# Autodesk Inventor assembly: NeckAssembly
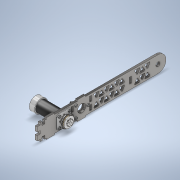
[picture p0: Inventor's stored thumbnail of the model, 180x180]
Saved by Autodesk Inventor 2022 (Build 260153000, 153)
## iProperties
Created: 2021-05-22
Part Number: NeckAssembly
Document SubType Name: Assembly
Designer: M3rob
Mass: 10239.7 g
Surface Area: 3396.39 cm^2
Volume: 1644.12 cm^3
Density: 6.22807 g/cm^3
Author: M3rob
## Documents named in this file (10)
- C:\Users\M3rob\Documents\GrabCAD\FireBird 250 Pound Gaming Machine\Drafts\FrameDrafts\Draft_04\Assemblies\NeckAssembly.iam
- C:\Users\M3rob\Documents\GrabCAD\FireBird 250 Pound Gaming Machine\Drafts\FrameDrafts\Draft_04\Chassis and Mounting\NeckFrame_Draft04.ipt
- C:\Users\M3rob\Documents\GrabCAD\FireBird 250 Pound Gaming Machine\Drafts\FrameDrafts\Draft_04\Chassis and Mounting\MotorMountingPlate_Draft02.ipt
- C:\Users\M3rob\Documents\GrabCAD\FireBird 250 Pound Gaming Machine\Drafts\FrameDrafts\Draft_04\Electronics\MagMotorMockup.ipt
- C:\Users\M3rob\Documents\GrabCAD\FireBird 250 Pound Gaming Machine\Drafts\FrameDrafts\Draft_04\Hardware\92620A656_GeneralChassisScrew.ipt
- C:\Users\M3rob\Documents\GrabCAD\FireBird 250 Pound Gaming Machine\Drafts\FrameDrafts\Draft_04\Hardware\94895A815_GeneralChassisNut.ipt
- C:\Users\M3rob\Documents\GrabCAD\FireBird 250 Pound Gaming Machine\Drafts\FrameDrafts\Draft_04\Hardware\2737T262_JackshaftSprocket_Modified.ipt
- C:\Users\M3rob\Documents\GrabCAD\FireBird 250 Pound Gaming Machine\Drafts\FrameDrafts\Draft_04\Weapon System\6524K421_TorqueLimiter.ipt
- C:\Users\M3rob\Documents\GrabCAD\FireBird 250 Pound Gaming Machine\Drafts\FrameDrafts\Draft_04\Hardware\91253A198_WeaponMotorMountingScrew.ipt
- C:\Users\M3rob\Documents\GrabCAD\FireBird 250 Pound Gaming Machine\Drafts\FrameDrafts\Draft_04\Weapon System\JackShaftRetentionPlate.ipt
## Components (24 placed, 9 different names)
1. NeckFrame_Draft04:1 — Mate:1, Mate:2, Mate:3, Mate:4, Mate:5, Mate:29, Mate:30, Mate:31, Mate:32, Mate:46, Mate:47, Mate:48, Mate:49, Mate:50, Mate:51, Mate:52
2. MotorMountingPlate_Draft02:1 — Mate:1, Mate:2, Mate:3, Mate:4, Mate:5, Mate:6, Mate:7, Mate:8, Mate:17, Mate:18, Mate:19, Mate:20, Mate:21, Mate:22, Mate:23, Mate:24, Mate:36, Mate:37, Mate:38, Mate:39, Flush:1, Flush:2, Flush:3, Flush:4, Mate:42
3. MagMotorMockup:1 — Mate:6, Mate:7, Mate:8, Mate:35
4. 92620A656_GeneralChassisScrew:1 — Mate:20, Mate:22, Mate:27
5. 94895A815_GeneralChassisNut:1 — Mate:28, Mate:29
6. 92620A656_GeneralChassisScrew:2 — Mate:19, Mate:21, Mate:25
7. 94895A815_GeneralChassisNut:2 — Mate:25, Mate:31
8. 92620A656_GeneralChassisScrew:3 — Mate:18, Mate:24, Mate:28
9. 94895A815_GeneralChassisNut:3 — Mate:27, Mate:30
10. 92620A656_GeneralChassisScrew:4 — Mate:17, Mate:23, Mate:26
11. 94895A815_GeneralChassisNut:4 — Mate:26, Mate:32
12. 2737T262_JackshaftSprocket_Modified:1 — Mate:34
13. 6524K421_TorqueLimiter:1 — Mate:34, Mate:35, Mate:42
14. 91253A198_WeaponMotorMountingScrew:1 — Mate:36, Flush:4
15. 91253A198_WeaponMotorMountingScrew:2 — Mate:37, Flush:3
16. 91253A198_WeaponMotorMountingScrew:3 — Mate:39, Flush:2
17. 91253A198_WeaponMotorMountingScrew:4 — Mate:38, Flush:1
18. JackShaftRetentionPlate:1 — Mate:46, Mate:47, Mate:48, Mate:49, Mate:53, Mate:54, Mate:55, Mate:56
19. 94895A815_GeneralChassisNut:5 — Flush:5, Flush:6
20. 92620A656_GeneralChassisScrew:5 — Mate:52, Mate:54
21. 94895A815_GeneralChassisNut:6 — Flush:5, Mate:56
22. 92620A656_GeneralChassisScrew:6 — Mate:51, Mate:55
23. 94895A815_GeneralChassisNut:7 — Flush:6
24. 92620A656_GeneralChassisScrew:7 — Mate:50, Mate:53
## Relationships (52: Mate 46, Flush 6)
- Mate:1: NeckFrame_Draft04:1 ↔ MotorMountingPlate_Draft02:1
- Mate:2: NeckFrame_Draft04:1 ↔ MotorMountingPlate_Draft02:1
- Mate:3: NeckFrame_Draft04:1 ↔ MotorMountingPlate_Draft02:1
- Mate:4: NeckFrame_Draft04:1 ↔ MotorMountingPlate_Draft02:1
- Mate:5: NeckFrame_Draft04:1 ↔ MotorMountingPlate_Draft02:1
- Mate:6: MotorMountingPlate_Draft02:1 ↔ MagMotorMockup:1
- Mate:7: MotorMountingPlate_Draft02:1 ↔ MagMotorMockup:1
- Mate:8: MotorMountingPlate_Draft02:1 ↔ MagMotorMockup:1
- Mate:17: MotorMountingPlate_Draft02:1 ↔ 92620A656_GeneralChassisScrew:4
- Mate:18: MotorMountingPlate_Draft02:1 ↔ 92620A656_GeneralChassisScrew:3
- Mate:19: MotorMountingPlate_Draft02:1 ↔ 92620A656_GeneralChassisScrew:2
- Mate:20: MotorMountingPlate_Draft02:1 ↔ 92620A656_GeneralChassisScrew:1
- Mate:21: MotorMountingPlate_Draft02:1 ↔ 92620A656_GeneralChassisScrew:2
- Mate:22: MotorMountingPlate_Draft02:1 ↔ 92620A656_GeneralChassisScrew:1
- Mate:23: MotorMountingPlate_Draft02:1 ↔ 92620A656_GeneralChassisScrew:4
- Mate:24: MotorMountingPlate_Draft02:1 ↔ 92620A656_GeneralChassisScrew:3
- Mate:25: 92620A656_GeneralChassisScrew:2 ↔ 94895A815_GeneralChassisNut:2
- Mate:26: 92620A656_GeneralChassisScrew:4 ↔ 94895A815_GeneralChassisNut:4
- Mate:27: 92620A656_GeneralChassisScrew:1 ↔ 94895A815_GeneralChassisNut:3
- Mate:28: 94895A815_GeneralChassisNut:1 ↔ 92620A656_GeneralChassisScrew:3
- Mate:29: NeckFrame_Draft04:1 ↔ 94895A815_GeneralChassisNut:1
- Mate:30: NeckFrame_Draft04:1 ↔ 94895A815_GeneralChassisNut:3
- Mate:31: NeckFrame_Draft04:1 ↔ 94895A815_GeneralChassisNut:2
- Mate:32: NeckFrame_Draft04:1 ↔ 94895A815_GeneralChassisNut:4
- [Mate]: 2737T262_JackshaftSprocket_Modified:1 ↔ 6524K421_TorqueLimiter:1
- Mate:34: 2737T262_JackshaftSprocket_Modified:1 ↔ 6524K421_TorqueLimiter:1
- Mate:35: MagMotorMockup:1 ↔ 6524K421_TorqueLimiter:1
- Mate:36: MotorMountingPlate_Draft02:1 ↔ 91253A198_WeaponMotorMountingScrew:1
- Mate:37: MotorMountingPlate_Draft02:1 ↔ 91253A198_WeaponMotorMountingScrew:2
- Mate:38: MotorMountingPlate_Draft02:1 ↔ 91253A198_WeaponMotorMountingScrew:4
- Mate:39: MotorMountingPlate_Draft02:1 ↔ 91253A198_WeaponMotorMountingScrew:3
- Flush:1: MotorMountingPlate_Draft02:1 ↔ 91253A198_WeaponMotorMountingScrew:4
- Flush:2: MotorMountingPlate_Draft02:1 ↔ 91253A198_WeaponMotorMountingScrew:3
- Flush:3: MotorMountingPlate_Draft02:1 ↔ 91253A198_WeaponMotorMountingScrew:2
- Flush:4: MotorMountingPlate_Draft02:1 ↔ 91253A198_WeaponMotorMountingScrew:1
- Mate:42 (23.8125 mm): MotorMountingPlate_Draft02:1 ↔ 6524K421_TorqueLimiter:1
- [Mate]: 94895A815_GeneralChassisNut:5 ↔ 92620A656_GeneralChassisScrew:5
- [Mate]: 94895A815_GeneralChassisNut:6 ↔ 92620A656_GeneralChassisScrew:6
- [Mate]: 94895A815_GeneralChassisNut:7 ↔ 92620A656_GeneralChassisScrew:7
- Mate:46: NeckFrame_Draft04:1 ↔ JackShaftRetentionPlate:1
- Mate:47: NeckFrame_Draft04:1 ↔ JackShaftRetentionPlate:1
- Mate:48: NeckFrame_Draft04:1 ↔ JackShaftRetentionPlate:1
- Mate:49: NeckFrame_Draft04:1 ↔ JackShaftRetentionPlate:1
- Mate:50: NeckFrame_Draft04:1 ↔ 92620A656_GeneralChassisScrew:7
- Mate:51: NeckFrame_Draft04:1 ↔ 92620A656_GeneralChassisScrew:6
- Mate:52: NeckFrame_Draft04:1 ↔ 92620A656_GeneralChassisScrew:5
- Flush:5: 94895A815_GeneralChassisNut:5 ↔ 94895A815_GeneralChassisNut:6
- Flush:6: 94895A815_GeneralChassisNut:5 ↔ 94895A815_GeneralChassisNut:7
- Mate:53: JackShaftRetentionPlate:1 ↔ 92620A656_GeneralChassisScrew:7
- Mate:54: JackShaftRetentionPlate:1 ↔ 92620A656_GeneralChassisScrew:5
- Mate:55: JackShaftRetentionPlate:1 ↔ 92620A656_GeneralChassisScrew:6
- Mate:56: JackShaftRetentionPlate:1 ↔ 94895A815_GeneralChassisNut:6
## Named parameters: d38_d5 = 0 mm, d39_d6 = 0 mm, d93_d30 = 0 mm, d94_d30 = 0 mm, d95_d30 = 0 mm
